# Autodesk Inventor assembly: SklopReduktora
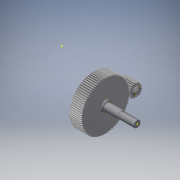
[picture p0: Inventor's stored thumbnail of the model, 180x180]
Saved by Autodesk Inventor 2018 (Build 220112000, 112)
## iProperties
Created: 2018-11-17
Part Number: SklopReduktora
Document SubType Name: Assembly
Designer: Kristijan
Author: Kristijan
## Documents named in this file (7)
- C:\Users\Kristijan\Dropbox\PolitehnikaPula\5 semestar\Konstrukcije\TimskiProjektniZadatak\OutputDrawings\SklopReduktora.iam
- C:\Users\Kristijan\Dropbox\PolitehnikaPula\5 semestar\Konstrukcije\TimskiProjektniZadatak\datasheetsModels\6008.iam
- C:\Users\Kristijan\Dropbox\PolitehnikaPula\5 semestar\Konstrukcije\TimskiProjektniZadatak\OutputDrawings\GonjenoVratilo.ipt
- C:\Users\Kristijan\Dropbox\PolitehnikaPula\5 semestar\Konstrukcije\TimskiProjektniZadatak\datasheetsModels\32913.iam
- C:\Users\Kristijan\Dropbox\PolitehnikaPula\5 semestar\Konstrukcije\TimskiProjektniZadatak\OutputDrawings\GonjeniZupcanik.ipt
- C:\Users\Kristijan\Dropbox\PolitehnikaPula\5 semestar\Konstrukcije\TimskiProjektniZadatak\datasheetsModels\DIN 6885 - A 22 x 14 x 90.ipt
- C:\Users\Kristijan\Dropbox\PolitehnikaPula\5 semestar\Konstrukcije\TimskiProjektniZadatak\OutputDrawings\PogonskoVratiloSaZupcanikom.ipt
## Components (8 placed, 6 different names)
1. 6008:1 [sub-assembly] — Mate:17, Mate:18
2. 6008:2 [sub-assembly] — Flush:14, Mate:15, Mate:16
3. GonjenoVratilo — Mate:6, Mate:7, Mate:8, Mate:9, udaljenostOsi, Mate:13, Rigid:1, Flush:15, Mate:14, Flush:16
4. 32913:1 [sub-assembly] — Mate:6, Mate:7, Flush:14
5. 32913:2 [sub-assembly] — Mate:8, Mate:9
6. GonjeniZupcanik — Mate:13, Flush:15, Mate:14, Rotation:1
7. DIN 6885-1 A A 22 x 14 x 90:1 — Rigid:1
8. Pogonsko vratilo sa zupcanikom — Mate:15, Mate:16, Mate:17, Mate:18, Flush:17, Rotation:1
## Relationships (17: Mate 11, Flush 4, WeldJoint 1, RelateRotation 1)
- Mate:6: GonjenoVratilo ↔ 32913:1
- Mate:7: GonjenoVratilo ↔ 32913:1
- Mate:8: GonjenoVratilo ↔ 32913:2
- Mate:9: GonjenoVratilo ↔ 32913:2
- udaljenostOsi [Mate] (262.5 mm): GonjenoVratilo
- Flush:14 (5 mm): 6008:2 ↔ 32913:1
- Mate:13: GonjenoVratilo ↔ GonjeniZupcanik
- Rigid:1 [WeldJoint]: GonjenoVratilo ↔ DIN 6885-1 A A 22 x 14 x 90:1
- Flush:15: GonjenoVratilo ↔ GonjeniZupcanik
- Mate:14: GonjenoVratilo ↔ GonjeniZupcanik
- Mate:15: 6008:2 ↔ Pogonsko vratilo sa zupcanikom
- Mate:16: 6008:2 ↔ Pogonsko vratilo sa zupcanikom
- Mate:17: 6008:1 ↔ Pogonsko vratilo sa zupcanikom
- Mate:18: 6008:1 ↔ Pogonsko vratilo sa zupcanikom
- Flush:16: GonjenoVratilo
- Flush:17: Pogonsko vratilo sa zupcanikom
- Rotation:1 [RelateRotation] (1 ul): GonjeniZupcanik ↔ Pogonsko vratilo sa zupcanikom
